# Autodesk Inventor assembly: Assembly
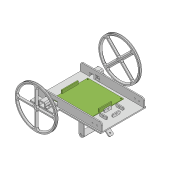
[picture p0: Inventor's stored thumbnail of the model, 180x180]
Saved by Autodesk Inventor 2017 (Build 210142000, 142)
## iProperties
Created: 2019-06-10
Part Number: Assembly
Document SubType Name: Assembly
Designer: markg
Author: markg
## Documents named in this file (8)
- C:\Users\markg\Documents\`School\`ME 433\Assignments&Workspaces\MarkGalperin_ME433_2019\HW16\CAD\Assembly.iam
- C:\Users\markg\Documents\`School\`ME 433\Assignments&Workspaces\MarkGalperin_ME433_2019\HW16\CAD\Chassis.ipt
- C:\Users\markg\Documents\`School\`ME 433\Assignments&Workspaces\MarkGalperin_ME433_2019\HW16\CAD\Board.ipt
- C:\Users\markg\Documents\`School\`ME 433\Assignments&Workspaces\MarkGalperin_ME433_2019\HW16\CAD\MotorCap.ipt
- C:\Users\markg\Documents\`School\`ME 433\Assignments&Workspaces\MarkGalperin_ME433_2019\HW16\CAD\Wheel.ipt
- C:\Users\markg\Documents\`School\`ME 433\Assignments&Workspaces\MarkGalperin_ME433_2019\HW16\CAD\batterywall.ipt
- C:\Users\markg\Documents\`School\`ME 433\Assignments&Workspaces\MarkGalperin_ME433_2019\HW16\CAD\wall.ipt
- C:\Users\markg\Documents\`School\`ME 433\Assignments&Workspaces\MarkGalperin_ME433_2019\HW16\CAD\spoonholder.ipt
## Components (13 placed, 7 different names)
1. Chassis:1 — Mate:3, Mate:4, Mate:5, Mate:6, Mate:7, Mate:12, Mate:13, Mate:14, Mate:15, Mate:16, Mate:17, Mate:18, Mate:19, Flush:1, Flush:2, Flush:3, Flush:4, Mate:20, Mate:21, Mate:22, Mate:23, Flush:5, Flush:6, Flush:7, Flush:8, Mate:24, Mate:25
2. Board:1 — Mate:3, Mate:4, Mate:5
3. MotorCap:1 — Mate:6, Mate:8, Mate:9, Mate:13, Mate:14
4. MotorCap:2 — Mate:7, Mate:10, Mate:11, Mate:12, Mate:15
5. Wheel:1 — Mate:10, Mate:11
6. Wheel:2 — Mate:8, Mate:9
7. batterywall:1 — Mate:16, Flush:2, Mate:22
8. batterywall:2 — Mate:18, Flush:3, Mate:21
9. batterywall:3 — Mate:19, Flush:4, Mate:23
10. batterywall:4 — Mate:17, Flush:1, Mate:20
11. wall:1 — Flush:5, Flush:7, Mate:25
12. wall:2 — Flush:6, Flush:8, Mate:24, Mate:26, Flush:9, Mate:27
13. spoonholder:1 — Mate:26, Flush:9, Mate:27
## Relationships (34: Mate 25, Flush 9)
- Mate:3: Chassis:1 ↔ Board:1
- Mate:4: Chassis:1 ↔ Board:1
- Mate:5: Chassis:1 ↔ Board:1
- Mate:6: Chassis:1 ↔ MotorCap:1
- Mate:7: Chassis:1 ↔ MotorCap:2
- Mate:8 (6.35 mm): MotorCap:1 ↔ Wheel:2
- Mate:9 (5.08 mm): MotorCap:1 ↔ Wheel:2
- Mate:10 (6.35 mm): MotorCap:2 ↔ Wheel:1
- Mate:11 (5.08 mm): MotorCap:2 ↔ Wheel:1
- Mate:12: Chassis:1 ↔ MotorCap:2
- Mate:13: Chassis:1 ↔ MotorCap:1
- Mate:14: Chassis:1 ↔ MotorCap:1
- Mate:15: Chassis:1 ↔ MotorCap:2
- Mate:16: Chassis:1 ↔ batterywall:1
- Mate:17: Chassis:1 ↔ batterywall:4
- Mate:18: Chassis:1 ↔ batterywall:2
- Mate:19: Chassis:1 ↔ batterywall:3
- Flush:1: Chassis:1 ↔ batterywall:4
- Flush:2: Chassis:1 ↔ batterywall:1
- Flush:3: Chassis:1 ↔ batterywall:2
- Flush:4: Chassis:1 ↔ batterywall:3
- Mate:20: Chassis:1 ↔ batterywall:4
- Mate:21: Chassis:1 ↔ batterywall:2
- Mate:22: Chassis:1 ↔ batterywall:1
- Mate:23: Chassis:1 ↔ batterywall:3
- Flush:5: Chassis:1 ↔ wall:1
- Flush:6: Chassis:1 ↔ wall:2
- Flush:7: Chassis:1 ↔ wall:1
- Flush:8: Chassis:1 ↔ wall:2
- Mate:24: Chassis:1 ↔ wall:2
- Mate:25: Chassis:1 ↔ wall:1
- Mate:26: wall:2 ↔ spoonholder:1
- Flush:9: wall:2 ↔ spoonholder:1
- Mate:27: wall:2 ↔ spoonholder:1
